# Autodesk Inventor assembly: angle_triangle_brace
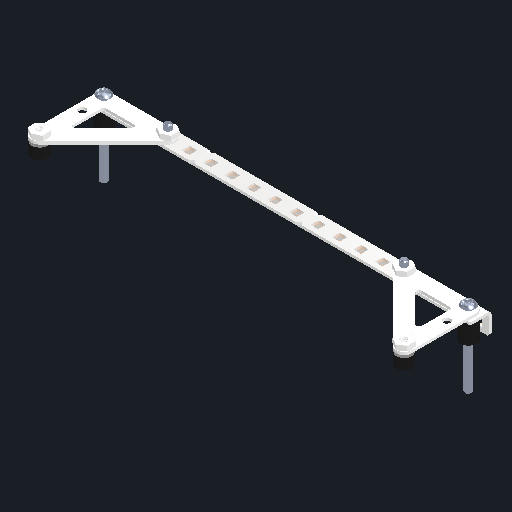
[picture p0: Inventor's stored thumbnail of the model, 512x512]
Saved by Autodesk Inventor 2025 (Build 290162000, 162)
## iProperties
Created: 2024-08-23
Part Number: angle_triangle_brace
Document SubType Name: Assembly
Designer: averey
Author: averey
## Documents named in this file (14)
- D:\vex_robotics_high_stakes\hardware\cad\bots\ENIGMA\chassis\drivetrain\structure\angle_triangle_brace.iam
- D:\vex_robotics_high_stakes\hardware\cad\ATLAS\chassis\structure\custom_parts\right_angle_gusset.ipt
- D:\vex_robotics_high_stakes\hardware\cad\VEX-CAD-Inventor\Structure\Angle\Aluminum 1x1\Alu Angle 1x1x18.ipt
- D:\vex_robotics_high_stakes\hardware\cad\VEX-CAD-Inventor\Structure\Hardware\Screw Shoulder Robosource\SScrew Shoulder Smooth .375 x .12.ipt
- C:\Users\avere\vex_robotics_high_stakes\hardware\cad\VEX-CAD-Inventor\Structure\Hardware\Screw Shoulder Robosource.ipt
- D:\vex_robotics_high_stakes\hardware\cad\VEX-CAD-Inventor\Structure\Hardware\Nut Nylon\Nut Nylon - White.ipt
- C:\Users\avere\vex_robotics_high_stakes\hardware\cad\VEX-CAD-Inventor\Structure\Hardware\Nut Nylon.ipt
- D:\vex_robotics_high_stakes\hardware\cad\VEX-CAD-Inventor\Motion\Spacers\Spacer Nylon .375 OD\NSpacer .375 OD x .500.ipt
- C:\Users\avere\vex_robotics_high_stakes\hardware\cad\VEX-CAD-Inventor\Motion\Spacers\Spacer Nylon .375 OD.ipt
- D:\vex_robotics_high_stakes\hardware\cad\VEX-CAD-Inventor\Motion\Spacers\Washer Steel\SWasher .375 OD x .062500.ipt
- C:\Users\avere\vex_robotics_high_stakes\hardware\cad\VEX-CAD-Inventor\Motion\Spacers\Washer Steel.ipt
- D:\vex_robotics_high_stakes\hardware\cad\VEX-CAD-Inventor\Structure\Hardware\Screw Steel - Star\SScrew Star Smooth 1.750.ipt
- C:\Users\avere\vex_robotics_high_stakes\hardware\cad\VEX-CAD-Inventor\Structure\Hardware\Screw Steel - Star.ipt
- D:\vex_robotics_high_stakes\hardware\cad\VEX-CAD-Inventor\Motion\Spacers\Spacer Nylon .375 OD\NSpacer .375 OD x .250.ipt
## Components (17 placed, 8 different names)
1. right_angle_gusset:1
2. right_angle_gusset:2
3. Alu Angle 1x1x18:1
4. SScrew Shoulder Smooth .375 x .12:1
5. Nut Nylon - White:1
6. NSpacer .375 OD x .500:1
7. NSpacer .375 OD x .500:2
8. SWasher .375 OD x .062500:1
9. SWasher .375 OD x .062500:2
10. Nut Nylon - White:2
11. Nut Nylon - White:3
12. Nut Nylon - White:4
13. SScrew Shoulder Smooth .375 x .12:2
14. SScrew Star Smooth 1.750:1
15. SScrew Star Smooth 1.750:2
16. NSpacer .375 OD x .250:3
17. NSpacer .375 OD x .250:4
## Relationships (18: Insert 16, Mate 2)
- [Insert] (-3.175 mm): right_angle_gusset:1 ↔ Alu Angle 1x1x18:1
- [Mate]: right_angle_gusset:2 ↔ Alu Angle 1x1x18:1
- [Insert]: right_angle_gusset:2 ↔ Alu Angle 1x1x18:1
- [Mate]: right_angle_gusset:1 ↔ Alu Angle 1x1x18:1
- [Insert]: Alu Angle 1x1x18:1 ↔ SScrew Shoulder Smooth .375 x .12:1
- [Insert]: right_angle_gusset:2 ↔ Nut Nylon - White:1
- [Insert]: Alu Angle 1x1x18:1 ↔ NSpacer .375 OD x .500:1
- [Insert]: Alu Angle 1x1x18:1 ↔ NSpacer .375 OD x .500:2
- [Insert]: right_angle_gusset:1 ↔ SWasher .375 OD x .062500:1
- [Insert]: right_angle_gusset:2 ↔ SWasher .375 OD x .062500:2
- [Insert]: right_angle_gusset:2 ↔ Nut Nylon - White:2
- [Insert]: right_angle_gusset:1 ↔ Nut Nylon - White:3
- [Insert]: right_angle_gusset:1 ↔ Nut Nylon - White:4
- [Insert]: Alu Angle 1x1x18:1 ↔ SScrew Shoulder Smooth .375 x .12:2
- [Insert] (1.5875 mm): right_angle_gusset:2 ↔ SScrew Star Smooth 1.750:1
- [Insert] (1.5875 mm): right_angle_gusset:1 ↔ SScrew Star Smooth 1.750:2
- [Insert]: SWasher .375 OD x .062500:2 ↔ NSpacer .375 OD x .250:3
- [Insert]: SWasher .375 OD x .062500:1 ↔ NSpacer .375 OD x .250:4
## Named parameters: d2_d6 = 0 mm, d5_d8 = 0 mm, d6_d13 = 0 mm, d7_d15 = 0 mm, d8_d17 = 0 mm
